# Autodesk Inventor assembly: MonoFilamentSpool
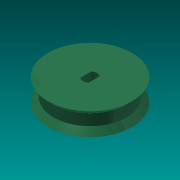
[picture p0: Inventor's stored thumbnail of the model, 180x180]
Saved by Autodesk Inventor 2013 (Build 170138000, 138)
## iProperties
Created: 2013-08-16
Part Number: MonoFilamentSpool
Document SubType Name: Assembly
Designer: Sawaiz
Author: Sawaiz
## Documents named in this file (3)
- S:\Sawaiz\Documents\3D Modeling\Inventor\PolarGraph\MonoFilamentSpool.iam
- S:\Sawaiz\Documents\3D Modeling\Inventor\PolarGraph\MonoFilamentSpoolFront.ipt
- S:\Sawaiz\Documents\3D Modeling\Inventor\PolarGraph\MonofilamentSpoolBack.ipt
## Components (2 placed, 2 different names)
1. MonoFilamentSpoolFront:1 — Insert:1, Mate:1
2. MonofilamentSpoolBack:1 — Insert:1, Mate:1
## Relationships (2: Insert 1, Mate 1)
- Insert:1: MonoFilamentSpoolFront:1 ↔ MonofilamentSpoolBack:1
- Mate:1: MonoFilamentSpoolFront:1 ↔ MonofilamentSpoolBack:1
